# Autodesk Inventor assembly: СборОчка
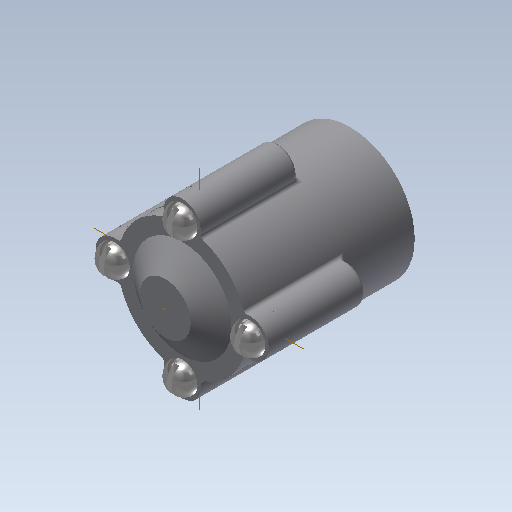
[picture p0: Inventor's stored thumbnail of the model, 512x512]
Saved by Autodesk Inventor 2021 (Build 250183000, 183)
## iProperties
Created: 2020-05-07
Part Number: СборОчка
Material: Типовые
Document SubType Name: Assembly
Designer: 2000
Mass: 388.771 g
Surface Area: 753.526 cm^2
Volume: 289.772 cm^3
Density: 1.34165 g/cm^3
Author: 2000
## Documents named in this file (4)
- C:\Users\2000\Desktop\СборОчка.iam
- C:\Users\2000\Desktop\Деталь1.ipt
- C:\Users\2000\Desktop\Деталь2.ipt
- C:\Users\2000\Documents\Inventor\Content Center Files\R2018\ru-RU\Screw B GOST 17473-80\Винт B.M12-6gx22 ГОСТ 17473-80.ipt
## Components (6 placed, 3 different names)
1. Деталь1:1 — С поворотом:1
2. Деталь2:1 — С поворотом:1, Вставка:1, Вставка:2, Вставка:3, Вставка:4
3. Винт B ГОСТ 17473-80 M12-6gx22:1 — Вставка:1
4. Винт B ГОСТ 17473-80 M12-6gx22:2 — Вставка:2
5. Винт B ГОСТ 17473-80 M12-6gx22:3 — Вставка:3
6. Винт B ГОСТ 17473-80 M12-6gx22:4 — Вставка:4
## Relationships (5: Insert 4, RevoluteJoint 1)
- С поворотом:1 [RevoluteJoint]: Деталь1:1 ↔ Деталь2:1
- Вставка:1 [Insert]: Деталь2:1 ↔ Винт B ГОСТ 17473-80 M12-6gx22:1
- Вставка:2 [Insert]: Деталь2:1 ↔ Винт B ГОСТ 17473-80 M12-6gx22:2
- Вставка:3 [Insert]: Деталь2:1 ↔ Винт B ГОСТ 17473-80 M12-6gx22:3
- Вставка:4 [Insert]: Деталь2:1 ↔ Винт B ГОСТ 17473-80 M12-6gx22:4
